# Autodesk Inventor assembly: glassMitSchutz
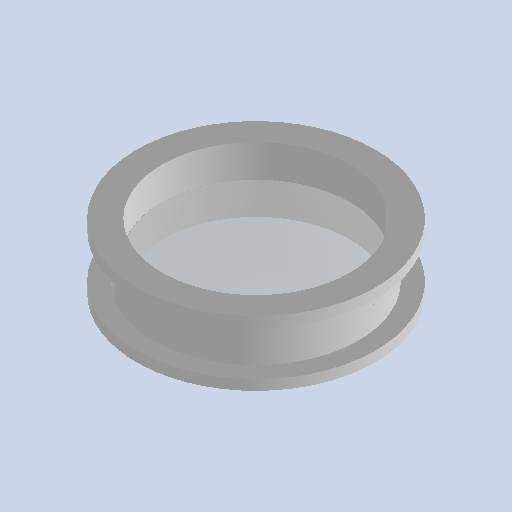
[picture p0: Inventor's stored thumbnail of the model, 512x512]
Saved by Autodesk Inventor 2025.1 (Build 291241000, 241)
## iProperties
Created: 2024-08-07
Part Number: glassMitSchutz
Document SubType Name: Assembly
Designer: ffogue
Author: ffogue
## Documents named in this file (3)
- C:\Users\ffogue\Documents\Inventor\BrandschutzTuer\glassMitSchutz.iam
- C:\Users\ffogue\Documents\Inventor\BrandschutzTuer\glass.ipt
- C:\Users\ffogue\Documents\Inventor\BrandschutzTuer\glassSchutz.ipt
## Components (3 placed, 2 different names)
1. glassSchutz:1 — Insert:1
2. glass:1 — Insert:1, Insert:2
3. glassSchutz:2 — Insert:2
## Relationships (2: Insert 2)
- Insert:1: glassSchutz:1 ↔ glass:1
- Insert:2: glass:1 ↔ glassSchutz:2
